# Autodesk Inventor assembly: Montagem2
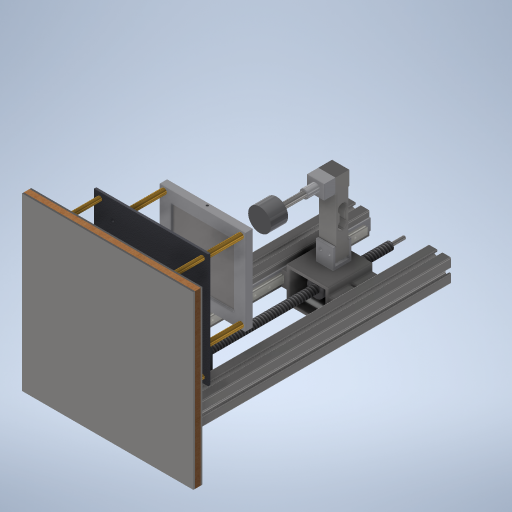
[picture p0: Inventor's stored thumbnail of the model, 512x512]
Saved by Autodesk Inventor 2023 (Build 270158000, 158)
## iProperties
Created: 2023-03-18
Part Number: Montagem2
Document SubType Name: Assembly
Designer: Mateus
Mass: 16088.3 g
Surface Area: 15425.7 cm^2
Volume: 3556.93 cm^3
Density: 4.52309 g/cm^3
Author: Mateus
## Documents named in this file (48)
- C:\Users\062190003\OneDrive\TCC\Desenho 3D\Montagem2.iam
- C:\Users\062190003\OneDrive\TCC\Desenho 3D\Base.ipt
- C:\Users\062190003\OneDrive\TCC\Desenho 3D\Fuso.ipt
- C:\Users\062190003\OneDrive\TCC\Desenho 3D\Motor.ipt
- C:\Users\062190003\OneDrive\TCC\Desenho 3D\Barra lateral.ipt
- C:\Users\062190003\OneDrive\TCC\Desenho 3D\Suporte 1.ipt
- C:\Users\062190003\OneDrive\TCC\Desenho 3D\Espaçador 1.ipt
- C:\Users\062190003\OneDrive\TCC\Desenho 3D\Espaçador 2.ipt
- C:\Users\062190003\OneDrive\TCC\Desenho 3D\Suporte 2.ipt
- C:\Users\062190003\OneDrive\TCC\Desenho 3D\Contra ponto.ipt
- C:\Users\062190003\OneDrive\TCC\Desenho 3D\Espaçador 3.ipt
- C:\Users\062190003\OneDrive\TCC\Desenho 3D\Mesa 1.ipt
- C:\Users\062190003\OneDrive\TCC\Desenho 3D\Guia.ipt
- C:\Users\062190003\OneDrive\TCC\Desenho 3D\Suporte guia.ipt
- C:\Users\062190003\OneDrive\TCC\Desenho 3D\Guia trilho.ipt
- C:\Users\062190003\OneDrive\TCC\Desenho 3D\Lado caixa 1.ipt
- C:\Users\062190003\OneDrive\TCC\Desenho 3D\Lado caixa 2.ipt
- C:\Users\062190003\OneDrive\TCC\Desenho 3D\Célula de carga 2.ipt
- C:\Users\062190003\OneDrive\TCC\Desenho 3D\Suporte braço 2.0.ipt
- C:\Users\062190003\OneDrive\TCC\Desenho 3D\Suporte ponta.ipt
- C:\Users\062190003\OneDrive\TCC\Desenho 3D\Trilho 2.ipt
- C:\Users\062190003\OneDrive\TCC\Desenho 3D\Mesa 2.ipt
- C:\Users\062190003\OneDrive\TCC\Desenho 3D\Espaçador 4.ipt
- C:\Users\062190003\OneDrive\TCC\Desenho 3D\Mesa 3.ipt
- C:\Users\062190003\OneDrive\TCC\Desenho 3D\Suporte mesa.ipt
- C:\Users\Mateus PC\Documents\Inventor\Content Center Files\R2023\pt-BR\BS 4168(1)\BS 4168 - M5 x 20(1).ipt
- C:\Users\Mateus PC\Documents\Inventor\Content Center Files\R2023\pt-BR\ANSI B18.3.1M(1)\ANSI B18.3.1M - M4x0,7 x 6(2).ipt
- C:\Users\Mateus PC\Documents\Inventor\Content Center Files\R2023\pt-BR\SKF - Single row ball bearings\SKF618_6.ipt
- C:\Users\Mateus PC\Documents\Inventor\Content Center Files\R2023\pt-BR\DIN 464\DIN 464 - M5 x 12.ipt
- C:\Users\Mateus PC\Documents\Inventor\Content Center Files\R2023\pt-BR\DIN 653\DIN 653 - M5 x 10.ipt
- C:\Users\Mateus PC\Documents\Inventor\Content Center Files\R2023\pt-BR\ISO 4762(2)\ISO 4762 - M4 x 35ISO.ipt
- C:\Users\Mateus PC\Documents\Inventor\Content Center Files\R2023\pt-BR\ISO 4032(2)\ISO 4032 - M4 - ISO.ipt
- C:\Users\Mateus PC\Documents\Inventor\Content Center Files\R2023\pt-BR\ISO 4762(2)\ISO 4762 - M4 x 6ISO.ipt
- C:\Users\Mateus PC\Documents\Inventor\Content Center Files\R2023\pt-BR\ISO 4762(2)\ISO 4762 - M4 x 8ISO.ipt
- C:\Users\Mateus PC\Documents\Inventor\Content Center Files\R2023\pt-BR\ISO 4762(2)\ISO 4762 - M5 x 35ISO.ipt
- C:\Users\Mateus PC\Documents\Inventor\Content Center Files\R2023\pt-BR\ISO 4762(2)\ISO 4762 - M2,5 x 8ISO.ipt
- C:\Users\Mateus PC\Documents\Inventor\Content Center Files\R2023\pt-BR\ISO 4762(2)\ISO 4762 - M2,5 x 10ISO.ipt
- C:\Users\062190003\OneDrive\TCC\Desenho 3D\Perfil aluminio.ipt
- C:\Users\Mateus PC\Documents\Inventor\Content Center Files\R2023\pt-BR\ISO 4762(2)\ISO 4762 - M4 x 16ISO.ipt
- C:\Users\062190003\OneDrive\TCC\Desenho 3D\Probe.ipt
- C:\Users\062190003\OneDrive\TCC\Desenho 3D\Base madeira.ipt
- C:\Users\Mateus PC\Documents\Inventor\Content Center Files\R2023\pt-BR\ISO 4762(2)\ISO 4762 - M3 x 30ISO.ipt
- C:\Users\062190003\OneDrive\TCC\Desenho 3D\Montagem2\AIP\FEA\eay7bn8rk.fins
- C:\Users\062190003\OneDrive\TCC\Desenho 3D\Montagem2\AIP\FEA\eay7bn8rk.fsat
- C:\Users\062190003\OneDrive\TCC\Desenho 3D\Montagem2\AIP\FEA\eay7bn8rk.ftes
- C:\Users\062190003\OneDrive\TCC\Desenho 3D\Montagem2\AIP\FEA\eay7bn8rk.fwiz
- C:\Users\062190003\OneDrive\TCC\Desenho 3D\Montagem2\AIP\FEA\eay7bn8xs.fmsh
- C:\Users\062190003\OneDrive\TCC\Desenho 3D\Montagem2\AIP\FEA\eay7bn8xt.fres
## Components (126 placed, 41 different names)
1. Base:1 — Coincidente:13, Alinhado:11, Coincidente:17, Alinhado:12, Coincidente:21, Coincidente:27, Coincidente:28, Coincidente:29, Coincidente:30, Coincidente:48, Alinhado:28, Alinhado:29, Coincidente:247, Alinhado:82, Coincidente:269, Alinhado:84, Coincidente:273, Alinhado:86
2. Fuso:1 — Coincidente:9, Coincidente:10, Coincidente:13, Coincidente:49, Coincidente:162, Coincidente:248
3. Motor:1 — Coincidente:9, Coincidente:10, Alinhado:11, Coincidente:24, Coincidente:25, Coincidente:26, Coincidente:40, Coincidente:184, Coincidente:185, Coincidente:186, Coincidente:187, Coincidente:188, Coincidente:189, Coincidente:190, Coincidente:191, Coincidente:193, Coincidente:195, Coincidente:197, Coincidente:199
4. Barra lateral:1 — Alinhado:16, Alinhado:17, Coincidente:245, Coincidente:251, Inserir:25, Inserir:26
5. Barra lateral:2 — Alinhado:16, Coincidente:21, Alinhado:17, Coincidente:246, Alinhado:79, Coincidente:250, Inserir:27, Inserir:28
6. Suporte 1:1 — Coincidente:24, Coincidente:25, Coincidente:26, Coincidente:31, Coincidente:32, Coincidente:33, Coincidente:34, Coincidente:35, Coincidente:36, Coincidente:37, Coincidente:38, Coincidente:39, Alinhado:22, Mate:117
7. Espaçador 1:1 — Coincidente:29, Coincidente:34, Mate:117
8. Espaçador 1:2 — Coincidente:27, Coincidente:33
9. Espaçador 1:3 — Coincidente:30, Coincidente:32
10. Espaçador 1:4 — Coincidente:28, Coincidente:31
11. Espaçador 2:1 — Coincidente:35, Alinhado:19, Alinhado:20, Coincidente:39, Coincidente:41
12. Espaçador 2:2 — Coincidente:36, Alinhado:20, Alinhado:21
13. Espaçador 2:3 — Coincidente:38, Alinhado:19
14. Espaçador 2:4 — Coincidente:37, Alinhado:21
15. Suporte 2:1 — Coincidente:40, Alinhado:22, Coincidente:41, Coincidente:148, Coincidente:149, Coincidente:150, Coincidente:151, Coincidente:152, Coincidente:153, Coincidente:154, Coincidente:155
16. Contra ponto:1 — Alinhado:71, Coincidente:248, Coincidente:252, Coincidente:253, Coincidente:254, Coincidente:255, Coincidente:256, Coincidente:257, Coincidente:258, Coincidente:259, Coincidente:260, Coincidente:261, Coincidente:262, Coincidente:263, Coincidente:264, Coincidente:265, Coincidente:266, Coincidente:267, Coincidente:268, Alinhado:83
17. Espaçador 3:1 — Coincidente:45, Alinhado:25, Alinhado:26
18. Espaçador 3:2 — Alinhado:25, Coincidente:47, Coincidente:48, Mate:119
19. Espaçador 3:3 — Coincidente:44, Alinhado:27
20. Espaçador 3:4 — Coincidente:43, Alinhado:26, Alinhado:27
21. Mesa 1:1 — Coincidente:43, Coincidente:44, Coincidente:45, Coincidente:47, Alinhado:28, Alinhado:29, Alinhado:61, Alinhado:62, Mate:119, Mate:121, Coincidente:160, Coincidente:161
22. Guia:1 — Coincidente:49, Coincidente:50, Coincidente:51
23. Suporte guia:1 — Coincidente:50, Coincidente:51, Coincidente:90, Alinhado:52, Coincidente:249
24. Guia trilho:1 — Mate:60, Coincidente:206, Alinhado:74
25. Guia trilho:2 — Mate:60, Flush:30, Coincidente:205, Alinhado:74, Coincidente:207, Alinhado:75, Coincidente:208
26. Guia trilho:3 — Mate:61, Alinhado:72, Alinhado:73
27. Guia trilho:4 — Mate:61, Flush:30, Coincidente:91, Alinhado:53, Alinhado:72, Alinhado:73, Coincidente:204, Alinhado:75, Alinhado:81
28. Lado caixa 1:2 — Alinhado:50, Alinhado:51, Coincidente:92, Mate:115, Flush:65, Coincidente:126, Coincidente:176, Coincidente:178, Coincidente:180, Coincidente:182
29. Lado caixa 2:2 — Coincidente:90, Coincidente:91, Alinhado:50, Alinhado:51, Coincidente:92, Alinhado:52, Alinhado:53, Coincidente:207, Coincidente:249, Alinhado:81
30. Célula de carga 2:1 — Coincidente:98, Alinhado:56, Alinhado:57, Flush:63, Flush:64, Mate:114, Coincidente:201, Coincidente:203
31. Suporte braço 2.0:1 — Flush:63, Flush:64, Mate:114, Mate:115, Flush:65, Coincidente:126, Inserir:5, Inserir:6, Coincidente:173, Coincidente:175, Coincidente:177, Coincidente:179, Coincidente:181, Coincidente:183
32. Suporte ponta:1 — Coincidente:98, Alinhado:56, Alinhado:57, Coincidente:200, Coincidente:202, Coincidente:270, Coincidente:271
33. Trilho 2:1 — Alinhado:58, Alinhado:59, Coincidente:205, Coincidente:206, Coincidente:208, Inserir:7, Inserir:8, Inserir:9, Inserir:10, Inserir:11, Inserir:12, Inserir:13, Inserir:14, Inserir:15, Inserir:16, Inserir:17, Inserir:18, Inserir:19, Inserir:20, Inserir:21, Inserir:22, Inserir:23, Inserir:24, Coincidente:251, Coincidente:269
34. Trilho 2:2 — Alinhado:58, Alinhado:59, Coincidente:204, Coincidente:209, Coincidente:210, Coincidente:211, Coincidente:212, Coincidente:213, Coincidente:214, Coincidente:215, Coincidente:216, Coincidente:217, Coincidente:218, Coincidente:219, Coincidente:220, Coincidente:221, Coincidente:222, Coincidente:223, Coincidente:224, Coincidente:225, Coincidente:226, Coincidente:227, Coincidente:228, Coincidente:229, Coincidente:230, Coincidente:231, Coincidente:232, Coincidente:233, Coincidente:234, Coincidente:235, Coincidente:236, Coincidente:237, Coincidente:238, Coincidente:239, Coincidente:240, Coincidente:241, Coincidente:242, Coincidente:243, Coincidente:244, Coincidente:250
35. Mesa 2:1 — Coincidente:106, Coincidente:107, Coincidente:108, Coincidente:109, Coincidente:110, Alinhado:61, Alinhado:62, Coincidente:111, Coincidente:112, Coincidente:113, Coincidente:136, Coincidente:138, Coincidente:140, Coincidente:142, Coincidente:167
36. Espaçador 4:1 — Coincidente:108, Flush:67, Flush:68, Mate:125, Coincidente:139
37. Espaçador 4:2 — Coincidente:106, Coincidente:110, Flush:68, Mate:123, Mate:124, Coincidente:137
38. Espaçador 4:3 — Coincidente:109, Flush:66, Flush:67, Coincidente:141
39. Espaçador 4:4 — Coincidente:107, Flush:66, Mate:122, Coincidente:135
40. Mesa 3:1 — Coincidente:111, Coincidente:112, Coincidente:113
41. Espaçador 3:5 — Coincidente:160, Coincidente:161
42. Suporte mesa:1 — Flush:69, Flush:70, Mate:121, Mate:122, Mate:123, Mate:124, Coincidente:163, Coincidente:164
43. Suporte mesa:2 — Flush:69, Flush:70, Mate:125, Coincidente:165, Coincidente:166
44. BS 4168 : Peça 1 Parafuso Allen de cabeça - Métrica M5 x 20:1 — Coincidente:135, Coincidente:136
45. BS 4168 : Peça 1 Parafuso Allen de cabeça - Métrica M5 x 20:2 — Coincidente:137, Coincidente:138
46. BS 4168 : Peça 1 Parafuso Allen de cabeça - Métrica M5 x 20:3 — Coincidente:139, Coincidente:140
47. BS 4168 : Peça 1 Parafuso Allen de cabeça - Métrica M5 x 20:4 — Coincidente:141, Coincidente:142
48. Parafuso Allen de cabeça escareada - Métrica M4x0,7 x 6:1 — Coincidente:148, Coincidente:149
49. Parafuso Allen de cabeça escareada - Métrica M4x0,7 x 6:2 — Coincidente:150, Coincidente:151
50. Parafuso Allen de cabeça escareada - Métrica M4x0,7 x 6:3 — Coincidente:152, Coincidente:153
51. Parafuso Allen de cabeça escareada - Métrica M4x0,7 x 6:4 — Coincidente:154, Coincidente:155
52. SKF- Mancais de esferas de fileira única SKF618/6:1 — Coincidente:162, Alinhado:71
53. DIN 464 M5 x 12:1 — Coincidente:163, Coincidente:164
54. DIN 464 M5 x 12:2 — Coincidente:165, Coincidente:166
55. DIN 653 M5 x 10:1 — Coincidente:167
56. ISO 4762 M4 x 35:1 — Inserir:5, Coincidente:174
57. ISO 4762 M4 x 35:2 — Inserir:6, Coincidente:172
58. ISO 4032 M4:1 — Coincidente:172, Coincidente:173
59. ISO 4032 M4:2 — Coincidente:174, Coincidente:175
60. ISO 4762 M4 x 6:1 — Coincidente:176, Coincidente:177
61. ISO 4762 M4 x 6:2 — Coincidente:178, Coincidente:179
62. ISO 4762 M4 x 6:3 — Coincidente:180, Coincidente:181
63. ISO 4762 M4 x 6:4 — Coincidente:182, Coincidente:183
64. ISO 4762 M4 x 8:1 — Coincidente:184, Coincidente:185, Coincidente:192
65. ISO 4762 M4 x 8:2 — Coincidente:186, Coincidente:187, Coincidente:194
66. ISO 4762 M4 x 8:3 — Coincidente:188, Coincidente:189, Coincidente:198
67. ISO 4762 M4 x 8:4 — Coincidente:190, Coincidente:191, Coincidente:196
68. ISO 4032 M4:3 — Coincidente:192, Coincidente:193
69. ISO 4032 M4:4 — Coincidente:194, Coincidente:195
70. ISO 4032 M4:5 — Coincidente:196, Coincidente:197
71. ISO 4032 M4:6 — Coincidente:198, Coincidente:199
72. ISO 4762 M5 x 35:1 — Coincidente:200, Coincidente:201
73. ISO 4762 M5 x 35:2 — Coincidente:202, Coincidente:203
74. ISO 4762 M2,5 x 8:1 — Inserir:7
75. ISO 4762 M2,5 x 8:2 — Inserir:8
76. ISO 4762 M2,5 x 8:3 — Inserir:9
77. ISO 4762 M2,5 x 8:4 — Inserir:10
78. ISO 4762 M2,5 x 8:5 — Inserir:11
79. ISO 4762 M2,5 x 8:6 — Inserir:12
80. ISO 4762 M2,5 x 8:7 — Inserir:13
81. ISO 4762 M2,5 x 8:8 — Inserir:14
82. ISO 4762 M2,5 x 8:9 — Inserir:15
83. ISO 4762 M2,5 x 8:10 — Inserir:16
84. ISO 4762 M2,5 x 8:11 — Inserir:17
85. ISO 4762 M2,5 x 8:12 — Inserir:18
86. ISO 4762 M2,5 x 8:13 — Inserir:19
87. ISO 4762 M2,5 x 8:14 — Inserir:20
88. ISO 4762 M2,5 x 8:15 — Inserir:21
89. ISO 4762 M2,5 x 8:16 — Inserir:22
90. ISO 4762 M2,5 x 8:17 — Inserir:23
91. ISO 4762 M2,5 x 8:18 — Inserir:24
92. ISO 4762 M2,5 x 10:1 — Coincidente:209, Coincidente:210
93. ISO 4762 M2,5 x 10:2 — Coincidente:211, Coincidente:212
94. ISO 4762 M2,5 x 10:3 — Coincidente:213, Coincidente:214
95. ISO 4762 M2,5 x 10:4 — Coincidente:215, Coincidente:216
96. ISO 4762 M2,5 x 10:5 — Coincidente:217, Coincidente:218
97. ISO 4762 M2,5 x 10:6 — Coincidente:219, Coincidente:220
98. ISO 4762 M2,5 x 10:7 — Coincidente:221, Coincidente:222
99. ISO 4762 M2,5 x 10:8 — Coincidente:223, Coincidente:224
100. ISO 4762 M2,5 x 10:9 — Coincidente:225, Coincidente:226
101. ISO 4762 M2,5 x 10:10 — Coincidente:227, Coincidente:228
102. ISO 4762 M2,5 x 10:11 — Coincidente:229, Coincidente:230
103. ISO 4762 M2,5 x 10:12 — Coincidente:231, Coincidente:232
104. ISO 4762 M2,5 x 10:13 — Coincidente:233, Coincidente:234
105. ISO 4762 M2,5 x 10:14 — Coincidente:235, Coincidente:236
106. ISO 4762 M2,5 x 10:15 — Coincidente:237, Coincidente:238
107. ISO 4762 M2,5 x 10:16 — Coincidente:239, Coincidente:240
108. ISO 4762 M2,5 x 10:17 — Coincidente:241, Coincidente:242
109. ISO 4762 M2,5 x 10:18 — Coincidente:243, Coincidente:244
110. Perfil aluminio:1 — Coincidente:246, Alinhado:77, Alinhado:78, Coincidente:247, Alinhado:79
111. Perfil aluminio:2 — Coincidente:245, Alinhado:77, Alinhado:78, Alinhado:82, Coincidente:252, Alinhado:83
112. ISO 4762 M4 x 16:1 — Coincidente:253, Coincidente:254
113. ISO 4762 M4 x 16:2 — Coincidente:255, Coincidente:256
114. ISO 4762 M4 x 16:3 — Coincidente:257, Coincidente:258
115. ISO 4762 M4 x 16:4 — Coincidente:259, Coincidente:260
116. ISO 4762 M4 x 16:5 — Coincidente:261, Coincidente:262
117. ISO 4762 M4 x 16:6 — Coincidente:263, Coincidente:264
118. ISO 4762 M4 x 16:7 — Coincidente:265, Coincidente:266
119. ISO 4762 M4 x 16:8 — Coincidente:267, Coincidente:268
120. Probe:1 — Coincidente:270, Coincidente:271
121. Base madeira:1 — Alinhado:84, Alinhado:85, Coincidente:272, Coincidente:273, Alinhado:86, Alinhado:87
122. Base:2 — Alinhado:85, Coincidente:272, Alinhado:87, Coincidente:274
123. ISO 4762 M3 x 30:1 — Inserir:25
124. ISO 4762 M3 x 30:2 — Inserir:26
125. ISO 4762 M3 x 30:3 — Inserir:27
126. ISO 4762 M3 x 30:4 — Inserir:28
## Relationships (253: Mate 182, Flush 47, Insert 24)
- Coincidente:9 [Mate] (0.5 mm): Fuso:1 ↔ Motor:1
- Coincidente:10 [Mate]: Fuso:1 ↔ Motor:1
- Coincidente:13 [Mate] (-150 mm): Base:1 ↔ Fuso:1
- Alinhado:11 [Flush] (20 mm): Base:1 ↔ Motor:1
- Coincidente:17 [Mate]: Base:1
- Alinhado:12 [Flush]: Base:1
- Alinhado:16 [Flush]: Barra lateral:1 ↔ Barra lateral:2
- Coincidente:21 [Mate]: Base:1 ↔ Barra lateral:2
- Alinhado:17 [Flush]: Barra lateral:1 ↔ Barra lateral:2
- Coincidente:24 [Mate]: Motor:1 ↔ Suporte 1:1
- Coincidente:25 [Mate]: Motor:1 ↔ Suporte 1:1
- Coincidente:26 [Mate]: Motor:1 ↔ Suporte 1:1
- Coincidente:27 [Mate]: Base:1 ↔ Espaçador 1:2
- Coincidente:28 [Mate]: Base:1 ↔ Espaçador 1:4
- Coincidente:29 [Mate]: Base:1 ↔ Espaçador 1:1
- Coincidente:30 [Mate]: Base:1 ↔ Espaçador 1:3
- Coincidente:31 [Mate]: Suporte 1:1 ↔ Espaçador 1:4
- Coincidente:32 [Mate]: Suporte 1:1 ↔ Espaçador 1:3
- Coincidente:33 [Mate]: Suporte 1:1 ↔ Espaçador 1:2
- Coincidente:34 [Mate]: Suporte 1:1 ↔ Espaçador 1:1
- Coincidente:35 [Mate]: Suporte 1:1 ↔ Espaçador 2:1
- Coincidente:36 [Mate]: Suporte 1:1 ↔ Espaçador 2:2
- Coincidente:37 [Mate]: Suporte 1:1 ↔ Espaçador 2:4
- Coincidente:38 [Mate]: Suporte 1:1 ↔ Espaçador 2:3
- Alinhado:19 [Flush]: Espaçador 2:1 ↔ Espaçador 2:3
- Alinhado:20 [Flush]: Espaçador 2:1 ↔ Espaçador 2:2
- Alinhado:21 [Flush]: Espaçador 2:2 ↔ Espaçador 2:4
- Coincidente:39 [Mate]: Suporte 1:1 ↔ Espaçador 2:1
- Coincidente:40 [Mate]: Motor:1 ↔ Suporte 2:1
- Alinhado:22 [Flush]: Suporte 1:1 ↔ Suporte 2:1
- Coincidente:41 [Mate]: Espaçador 2:1 ↔ Suporte 2:1
- Coincidente:43 [Mate]: Espaçador 3:4 ↔ Mesa 1:1
- Coincidente:44 [Mate]: Espaçador 3:3 ↔ Mesa 1:1
- Coincidente:45 [Mate]: Espaçador 3:1 ↔ Mesa 1:1
- Alinhado:25 [Flush]: Espaçador 3:1 ↔ Espaçador 3:2
- Alinhado:26 [Flush]: Espaçador 3:1 ↔ Espaçador 3:4
- Alinhado:27 [Flush]: Espaçador 3:3 ↔ Espaçador 3:4
- Coincidente:47 [Mate]: Espaçador 3:2 ↔ Mesa 1:1
- Coincidente:48 [Mate]: Base:1 ↔ Espaçador 3:2
- Alinhado:28 [Flush] (50 mm): Base:1 ↔ Mesa 1:1
- Alinhado:29 [Flush] (5.8 mm): Base:1 ↔ Mesa 1:1
- Coincidente:49 [Mate]: Fuso:1 ↔ Guia:1
- Coincidente:50 [Mate]: Guia:1 ↔ Suporte guia:1
- Coincidente:51 [Mate]: Guia:1 ↔ Suporte guia:1
- Mate:60 (5 mm): Guia trilho:1 ↔ Guia trilho:2
- Mate:61 (5 mm): Guia trilho:3 ↔ Guia trilho:4
- Flush:30: Guia trilho:2 ↔ Guia trilho:4
- Coincidente:90 [Mate]: Suporte guia:1 ↔ Lado caixa 2:2
- Coincidente:91 [Mate]: Guia trilho:4 ↔ Lado caixa 2:2
- Alinhado:50 [Flush]: Lado caixa 1:2 ↔ Lado caixa 2:2
- Alinhado:51 [Flush]: Lado caixa 1:2 ↔ Lado caixa 2:2
- Coincidente:92 [Mate]: Lado caixa 1:2 ↔ Lado caixa 2:2
- Alinhado:52 [Flush] (-21.5 mm): Suporte guia:1 ↔ Lado caixa 2:2
- Alinhado:53 [Flush] (-0.75 mm): Guia trilho:4 ↔ Lado caixa 2:2
- Coincidente:98 [Mate]: Célula de carga 2:1 ↔ Suporte ponta:1
- Alinhado:56 [Flush]: Célula de carga 2:1 ↔ Suporte ponta:1
- Alinhado:57 [Flush]: Célula de carga 2:1 ↔ Suporte ponta:1
- Alinhado:58 [Flush]: Trilho 2:1 ↔ Trilho 2:2
- Alinhado:59 [Flush]: Trilho 2:1 ↔ Trilho 2:2
- Coincidente:106 [Mate]: Mesa 2:1 ↔ Espaçador 4:2
- Coincidente:107 [Mate]: Mesa 2:1 ↔ Espaçador 4:4
- Coincidente:108 [Mate]: Mesa 2:1 ↔ Espaçador 4:1
- Coincidente:109 [Mate]: Mesa 2:1 ↔ Espaçador 4:3
- Coincidente:110 [Mate]: Mesa 2:1 ↔ Espaçador 4:2
- Alinhado:61 [Flush] (25 mm): Mesa 1:1 ↔ Mesa 2:1
- Alinhado:62 [Flush] (25 mm): Mesa 1:1 ↔ Mesa 2:1
- Coincidente:111 [Mate]: Mesa 2:1 ↔ Mesa 3:1
- Coincidente:112 [Mate]: Mesa 2:1 ↔ Mesa 3:1
- Coincidente:113 [Mate]: Mesa 2:1 ↔ Mesa 3:1
- Flush:63: Célula de carga 2:1 ↔ Suporte braço 2.0:1
- Flush:64: Célula de carga 2:1 ↔ Suporte braço 2.0:1
- Mate:114: Célula de carga 2:1 ↔ Suporte braço 2.0:1
- Mate:115: Lado caixa 1:2 ↔ Suporte braço 2.0:1
- Flush:65 (15 mm): Lado caixa 1:2 ↔ Suporte braço 2.0:1
- Mate:117: Suporte 1:1 ↔ Espaçador 1:1
- Mate:119: Espaçador 3:2 ↔ Mesa 1:1
- Flush:66: Espaçador 4:3 ↔ Espaçador 4:4
- Flush:67: Espaçador 4:1 ↔ Espaçador 4:3
- Flush:68: Espaçador 4:1 ↔ Espaçador 4:2
- Flush:69: Suporte mesa:1 ↔ Suporte mesa:2
- Flush:70: Suporte mesa:1 ↔ Suporte mesa:2
- Mate:121: Mesa 1:1 ↔ Suporte mesa:1
- Mate:122: Espaçador 4:4 ↔ Suporte mesa:1
- Mate:123: Espaçador 4:2 ↔ Suporte mesa:1
- Mate:124: Espaçador 4:2 ↔ Suporte mesa:1
- Mate:125: Espaçador 4:1 ↔ Suporte mesa:2
- Coincidente:126 [Mate]: Lado caixa 1:2 ↔ Suporte braço 2.0:1
- Coincidente:135 [Mate]: Espaçador 4:4 ↔ BS 4168 : Peça 1 Parafuso Allen de cabeça - Métrica M5 x 20:1
- Coincidente:136 [Mate]: Mesa 2:1 ↔ BS 4168 : Peça 1 Parafuso Allen de cabeça - Métrica M5 x 20:1
- Coincidente:137 [Mate]: Espaçador 4:2 ↔ BS 4168 : Peça 1 Parafuso Allen de cabeça - Métrica M5 x 20:2
- Coincidente:138 [Mate]: Mesa 2:1 ↔ BS 4168 : Peça 1 Parafuso Allen de cabeça - Métrica M5 x 20:2
- Coincidente:139 [Mate]: Espaçador 4:1 ↔ BS 4168 : Peça 1 Parafuso Allen de cabeça - Métrica M5 x 20:3
- Coincidente:140 [Mate]: Mesa 2:1 ↔ BS 4168 : Peça 1 Parafuso Allen de cabeça - Métrica M5 x 20:3
- Coincidente:141 [Mate]: Espaçador 4:3 ↔ BS 4168 : Peça 1 Parafuso Allen de cabeça - Métrica M5 x 20:4
- Coincidente:142 [Mate]: Mesa 2:1 ↔ BS 4168 : Peça 1 Parafuso Allen de cabeça - Métrica M5 x 20:4
- Coincidente:148 [Mate]: Suporte 2:1 ↔ Parafuso Allen de cabeça escareada - Métrica M4x0,7 x 6:1
- Coincidente:149 [Mate]: Suporte 2:1 ↔ Parafuso Allen de cabeça escareada - Métrica M4x0,7 x 6:1
- Coincidente:150 [Mate]: Suporte 2:1 ↔ Parafuso Allen de cabeça escareada - Métrica M4x0,7 x 6:2
- Coincidente:151 [Mate]: Suporte 2:1 ↔ Parafuso Allen de cabeça escareada - Métrica M4x0,7 x 6:2
- Coincidente:152 [Mate]: Suporte 2:1 ↔ Parafuso Allen de cabeça escareada - Métrica M4x0,7 x 6:3
- Coincidente:153 [Mate]: Suporte 2:1 ↔ Parafuso Allen de cabeça escareada - Métrica M4x0,7 x 6:3
- Coincidente:154 [Mate]: Suporte 2:1 ↔ Parafuso Allen de cabeça escareada - Métrica M4x0,7 x 6:4
- Coincidente:155 [Mate]: Suporte 2:1 ↔ Parafuso Allen de cabeça escareada - Métrica M4x0,7 x 6:4
- Coincidente:160 [Mate]: Mesa 1:1 ↔ Espaçador 3:5
- Coincidente:161 [Mate]: Mesa 1:1 ↔ Espaçador 3:5
- Coincidente:162 [Mate]: Fuso:1 ↔ SKF- Mancais de esferas de fileira única SKF618/6:1
- Alinhado:71 [Flush] (1 mm): Contra ponto:1 ↔ SKF- Mancais de esferas de fileira única SKF618/6:1
- Coincidente:163 [Mate]: Suporte mesa:1 ↔ DIN 464 M5 x 12:1
- Coincidente:164 [Mate]: Suporte mesa:1 ↔ DIN 464 M5 x 12:1
- Coincidente:165 [Mate]: Suporte mesa:2 ↔ DIN 464 M5 x 12:2
- Coincidente:166 [Mate]: Suporte mesa:2 ↔ DIN 464 M5 x 12:2
- Coincidente:167 [Mate]: Mesa 2:1 ↔ DIN 653 M5 x 10:1
- Inserir:5: Suporte braço 2.0:1 ↔ ISO 4762 M4 x 35:1
- Inserir:6: Suporte braço 2.0:1 ↔ ISO 4762 M4 x 35:2
- Coincidente:172 [Mate]: ISO 4762 M4 x 35:2 ↔ ISO 4032 M4:1
- Coincidente:173 [Mate]: Suporte braço 2.0:1 ↔ ISO 4032 M4:1
- Coincidente:174 [Mate]: ISO 4762 M4 x 35:1 ↔ ISO 4032 M4:2
- Coincidente:175 [Mate]: Suporte braço 2.0:1 ↔ ISO 4032 M4:2
- Coincidente:176 [Mate]: Lado caixa 1:2 ↔ ISO 4762 M4 x 6:1
- Coincidente:177 [Mate]: Suporte braço 2.0:1 ↔ ISO 4762 M4 x 6:1
- Coincidente:178 [Mate]: Lado caixa 1:2 ↔ ISO 4762 M4 x 6:2
- Coincidente:179 [Mate]: Suporte braço 2.0:1 ↔ ISO 4762 M4 x 6:2
- Coincidente:180 [Mate]: Lado caixa 1:2 ↔ ISO 4762 M4 x 6:3
- Coincidente:181 [Mate]: Suporte braço 2.0:1 ↔ ISO 4762 M4 x 6:3
- Coincidente:182 [Mate]: Lado caixa 1:2 ↔ ISO 4762 M4 x 6:4
- Coincidente:183 [Mate]: Suporte braço 2.0:1 ↔ ISO 4762 M4 x 6:4
- Coincidente:184 [Mate]: Motor:1 ↔ ISO 4762 M4 x 8:1
- Coincidente:185 [Mate]: Motor:1 ↔ ISO 4762 M4 x 8:1
- Coincidente:186 [Mate]: Motor:1 ↔ ISO 4762 M4 x 8:2
- Coincidente:187 [Mate]: Motor:1 ↔ ISO 4762 M4 x 8:2
- Coincidente:188 [Mate]: Motor:1 ↔ ISO 4762 M4 x 8:3
- Coincidente:189 [Mate]: Motor:1 ↔ ISO 4762 M4 x 8:3
- Coincidente:190 [Mate]: Motor:1 ↔ ISO 4762 M4 x 8:4
- Coincidente:191 [Mate]: Motor:1 ↔ ISO 4762 M4 x 8:4
- Coincidente:192 [Mate]: ISO 4762 M4 x 8:1 ↔ ISO 4032 M4:3
- Coincidente:193 [Mate]: Motor:1 ↔ ISO 4032 M4:3
- Coincidente:194 [Mate]: ISO 4762 M4 x 8:2 ↔ ISO 4032 M4:4
- Coincidente:195 [Mate]: Motor:1 ↔ ISO 4032 M4:4
- Coincidente:196 [Mate]: ISO 4762 M4 x 8:4 ↔ ISO 4032 M4:5
- Coincidente:197 [Mate]: Motor:1 ↔ ISO 4032 M4:5
- Coincidente:198 [Mate]: ISO 4762 M4 x 8:3 ↔ ISO 4032 M4:6
- Coincidente:199 [Mate]: Motor:1 ↔ ISO 4032 M4:6
- Coincidente:200 [Mate]: Suporte ponta:1 ↔ ISO 4762 M5 x 35:1
- Coincidente:201 [Mate]: Célula de carga 2:1 ↔ ISO 4762 M5 x 35:1
- Coincidente:202 [Mate]: Suporte ponta:1 ↔ ISO 4762 M5 x 35:2
- Coincidente:203 [Mate]: Célula de carga 2:1 ↔ ISO 4762 M5 x 35:2
- Alinhado:72 [Flush]: Guia trilho:3 ↔ Guia trilho:4
- Alinhado:73 [Flush]: Guia trilho:3 ↔ Guia trilho:4
- Coincidente:204 [Mate]: Guia trilho:4 ↔ Trilho 2:2
- Coincidente:205 [Mate]: Guia trilho:2 ↔ Trilho 2:1
- Coincidente:206 [Mate]: Guia trilho:1 ↔ Trilho 2:1
- Alinhado:74 [Flush]: Guia trilho:1 ↔ Guia trilho:2
- Coincidente:207 [Mate]: Guia trilho:2 ↔ Lado caixa 2:2
- Alinhado:75 [Flush]: Guia trilho:2 ↔ Guia trilho:4
- Coincidente:208 [Mate]: Guia trilho:2 ↔ Trilho 2:1
- Inserir:7: Trilho 2:1 ↔ ISO 4762 M2,5 x 8:1
- Inserir:8: Trilho 2:1 ↔ ISO 4762 M2,5 x 8:2
- Inserir:9: Trilho 2:1 ↔ ISO 4762 M2,5 x 8:3
- Inserir:10: Trilho 2:1 ↔ ISO 4762 M2,5 x 8:4
- Inserir:11: Trilho 2:1 ↔ ISO 4762 M2,5 x 8:5
- Inserir:12: Trilho 2:1 ↔ ISO 4762 M2,5 x 8:6
- Inserir:13: Trilho 2:1 ↔ ISO 4762 M2,5 x 8:7
- Inserir:14: Trilho 2:1 ↔ ISO 4762 M2,5 x 8:8
- Inserir:15: Trilho 2:1 ↔ ISO 4762 M2,5 x 8:9
- Inserir:16: Trilho 2:1 ↔ ISO 4762 M2,5 x 8:10
- Inserir:17: Trilho 2:1 ↔ ISO 4762 M2,5 x 8:11
- Inserir:18: Trilho 2:1 ↔ ISO 4762 M2,5 x 8:12
- Inserir:19: Trilho 2:1 ↔ ISO 4762 M2,5 x 8:13
- Inserir:20: Trilho 2:1 ↔ ISO 4762 M2,5 x 8:14
- Inserir:21: Trilho 2:1 ↔ ISO 4762 M2,5 x 8:15
- Inserir:22: Trilho 2:1 ↔ ISO 4762 M2,5 x 8:16
- Inserir:23: Trilho 2:1 ↔ ISO 4762 M2,5 x 8:17
- Inserir:24: Trilho 2:1 ↔ ISO 4762 M2,5 x 8:18
- Coincidente:209 [Mate]: Trilho 2:2 ↔ ISO 4762 M2,5 x 10:1
- Coincidente:210 [Mate]: Trilho 2:2 ↔ ISO 4762 M2,5 x 10:1
- Coincidente:211 [Mate]: Trilho 2:2 ↔ ISO 4762 M2,5 x 10:2
- Coincidente:212 [Mate]: Trilho 2:2 ↔ ISO 4762 M2,5 x 10:2
- Coincidente:213 [Mate]: Trilho 2:2 ↔ ISO 4762 M2,5 x 10:3
- Coincidente:214 [Mate]: Trilho 2:2 ↔ ISO 4762 M2,5 x 10:3
- Coincidente:215 [Mate]: Trilho 2:2 ↔ ISO 4762 M2,5 x 10:4
- Coincidente:216 [Mate]: Trilho 2:2 ↔ ISO 4762 M2,5 x 10:4
- Coincidente:217 [Mate]: Trilho 2:2 ↔ ISO 4762 M2,5 x 10:5
- Coincidente:218 [Mate]: Trilho 2:2 ↔ ISO 4762 M2,5 x 10:5
- Coincidente:219 [Mate]: Trilho 2:2 ↔ ISO 4762 M2,5 x 10:6
- Coincidente:220 [Mate]: Trilho 2:2 ↔ ISO 4762 M2,5 x 10:6
- Coincidente:221 [Mate]: Trilho 2:2 ↔ ISO 4762 M2,5 x 10:7
- Coincidente:222 [Mate]: Trilho 2:2 ↔ ISO 4762 M2,5 x 10:7
- Coincidente:223 [Mate]: Trilho 2:2 ↔ ISO 4762 M2,5 x 10:8
- Coincidente:224 [Mate]: Trilho 2:2 ↔ ISO 4762 M2,5 x 10:8
- Coincidente:225 [Mate]: Trilho 2:2 ↔ ISO 4762 M2,5 x 10:9
- Coincidente:226 [Mate]: Trilho 2:2 ↔ ISO 4762 M2,5 x 10:9
- Coincidente:227 [Mate]: Trilho 2:2 ↔ ISO 4762 M2,5 x 10:10
- Coincidente:228 [Mate]: Trilho 2:2 ↔ ISO 4762 M2,5 x 10:10
- Coincidente:229 [Mate]: Trilho 2:2 ↔ ISO 4762 M2,5 x 10:11
- Coincidente:230 [Mate]: Trilho 2:2 ↔ ISO 4762 M2,5 x 10:11
- Coincidente:231 [Mate]: Trilho 2:2 ↔ ISO 4762 M2,5 x 10:12
- Coincidente:232 [Mate]: Trilho 2:2 ↔ ISO 4762 M2,5 x 10:12
- Coincidente:233 [Mate]: Trilho 2:2 ↔ ISO 4762 M2,5 x 10:13
- Coincidente:234 [Mate]: Trilho 2:2 ↔ ISO 4762 M2,5 x 10:13
- Coincidente:235 [Mate]: Trilho 2:2 ↔ ISO 4762 M2,5 x 10:14
- Coincidente:236 [Mate]: Trilho 2:2 ↔ ISO 4762 M2,5 x 10:14
- Coincidente:237 [Mate]: Trilho 2:2 ↔ ISO 4762 M2,5 x 10:15
- Coincidente:238 [Mate]: Trilho 2:2 ↔ ISO 4762 M2,5 x 10:15
- Coincidente:239 [Mate]: Trilho 2:2 ↔ ISO 4762 M2,5 x 10:16
- Coincidente:240 [Mate]: Trilho 2:2 ↔ ISO 4762 M2,5 x 10:16
- Coincidente:241 [Mate]: Trilho 2:2 ↔ ISO 4762 M2,5 x 10:17
- Coincidente:242 [Mate]: Trilho 2:2 ↔ ISO 4762 M2,5 x 10:17
- Coincidente:243 [Mate]: Trilho 2:2 ↔ ISO 4762 M2,5 x 10:18
- Coincidente:244 [Mate]: Trilho 2:2 ↔ ISO 4762 M2,5 x 10:18
- Coincidente:245 [Mate]: Barra lateral:1 ↔ Perfil aluminio:2
- Coincidente:246 [Mate]: Barra lateral:2 ↔ Perfil aluminio:1
- Alinhado:77 [Flush]: Perfil aluminio:1 ↔ Perfil aluminio:2
- Alinhado:78 [Flush]: Perfil aluminio:1 ↔ Perfil aluminio:2
- Coincidente:247 [Mate]: Base:1 ↔ Perfil aluminio:1
- Coincidente:248 [Mate]: Fuso:1 ↔ Contra ponto:1
- Coincidente:249 [Mate] (11.5 mm): Suporte guia:1 ↔ Lado caixa 2:2
- Alinhado:79 [Flush] (-10 mm): Barra lateral:2 ↔ Perfil aluminio:1
- Coincidente:250 [Mate]: Barra lateral:2 ↔ Trilho 2:2
- Coincidente:251 [Mate]: Barra lateral:1 ↔ Trilho 2:1
- Alinhado:81 [Flush] (-21.5 mm): Guia trilho:4 ↔ Lado caixa 2:2
- Alinhado:82 [Flush] (28.4 mm): Base:1 ↔ Perfil aluminio:2
- Coincidente:252 [Mate]: Contra ponto:1 ↔ Perfil aluminio:2
- Coincidente:253 [Mate]: Contra ponto:1 ↔ ISO 4762 M4 x 16:1
- Coincidente:254 [Mate]: Contra ponto:1 ↔ ISO 4762 M4 x 16:1
- Coincidente:255 [Mate]: Contra ponto:1 ↔ ISO 4762 M4 x 16:2
- Coincidente:256 [Mate]: Contra ponto:1 ↔ ISO 4762 M4 x 16:2
- Coincidente:257 [Mate]: Contra ponto:1 ↔ ISO 4762 M4 x 16:3
- Coincidente:258 [Mate]: Contra ponto:1 ↔ ISO 4762 M4 x 16:3
- Coincidente:259 [Mate]: Contra ponto:1 ↔ ISO 4762 M4 x 16:4
- Coincidente:260 [Mate]: Contra ponto:1 ↔ ISO 4762 M4 x 16:4
- Coincidente:261 [Mate]: Contra ponto:1 ↔ ISO 4762 M4 x 16:5
- Coincidente:262 [Mate]: Contra ponto:1 ↔ ISO 4762 M4 x 16:5
- Coincidente:263 [Mate]: Contra ponto:1 ↔ ISO 4762 M4 x 16:6
- Coincidente:264 [Mate]: Contra ponto:1 ↔ ISO 4762 M4 x 16:6
- Coincidente:265 [Mate]: Contra ponto:1 ↔ ISO 4762 M4 x 16:7
- Coincidente:266 [Mate]: Contra ponto:1 ↔ ISO 4762 M4 x 16:7
- Coincidente:267 [Mate]: Contra ponto:1 ↔ ISO 4762 M4 x 16:8
- Coincidente:268 [Mate]: Contra ponto:1 ↔ ISO 4762 M4 x 16:8
- Alinhado:83 [Flush]: Contra ponto:1 ↔ Perfil aluminio:2
- Coincidente:269 [Mate] (12.5 mm): Base:1 ↔ Trilho 2:1
- Coincidente:270 [Mate]: Suporte ponta:1 ↔ Probe:1
- Coincidente:271 [Mate] (2 mm): Suporte ponta:1 ↔ Probe:1
- Alinhado:84 [Flush]: Base:1 ↔ Base madeira:1
- Alinhado:85 [Flush]: Base madeira:1 ↔ Base:2
- Coincidente:272 [Mate]: Base madeira:1 ↔ Base:2
- Coincidente:273 [Mate]: Base:1 ↔ Base madeira:1
- Alinhado:86 [Flush]: Base:1 ↔ Base madeira:1
- Alinhado:87 [Flush]: Base madeira:1 ↔ Base:2
- Inserir:25: Barra lateral:1 ↔ ISO 4762 M3 x 30:1
- Inserir:26: Barra lateral:1 ↔ ISO 4762 M3 x 30:2
- Inserir:27: Barra lateral:2 ↔ ISO 4762 M3 x 30:3
- Inserir:28: Barra lateral:2 ↔ ISO 4762 M3 x 30:4
- Coincidente:274 [Mate]: Base:2
## Named parameters: sa_1 = 10000, sa_0 = 10000
note: some values were not read from the file. Shown as the stored number, unit unknown: "sa_1", "sa_0".
